# Autodesk Inventor assembly: Передача с помощью зубчатых ремней
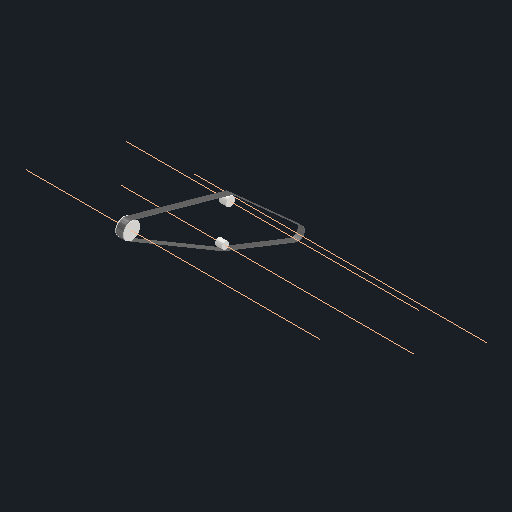
[picture p0: Inventor's stored thumbnail of the model, 512x512]
Saved by Autodesk Inventor 2024 (Build 280153000, 153)
## iProperties
ClientObjectVersion: 1
Created: 2023-09-26
Part Number: Передача с помощью зубчатых ремней
Document SubType Name: Assembly
Designer: user
Author: user
## Documents named in this file (5)
- D:\Docs\Robot\3d_v2\main_assembly\Мастер проектирования\Передача с помощью зубчатых ремней1.iam
- D:\Docs\Robot\3d_v2\main_assembly\Мастер проектирования\Зубчатый ремень1.ipt
- D:\Docs\Robot\3d_v2\main_assembly\Мастер проектирования\Шкив гладкий11.ipt
- D:\Docs\Robot\3d_v2\main_assembly\Мастер проектирования\Синхронный шкив21.ipt
- D:\Docs\Robot\3d_v2\main_assembly\Мастер проектирования\Шкив гладкий21.ipt
## Components (4 placed, 4 different names)
1. Зубчатый ремень:1 — Заподлицо:1, Совмещение:1, Заподлицо:2, Совмещение:2, Совмещение:3, Заподлицо:3, Совмещение:4
2. Шкив гладкий1:1 — Заподлицо:1, Совмещение:1
3. Синхронный шкив2:1 — Заподлицо:2, Совмещение:2, Совмещение:3
4. Шкив гладкий2:1 — Заподлицо:3, Совмещение:4
## Relationships (7: Mate 4, Flush 3)
- Заподлицо:1 [Flush]: Зубчатый ремень:1 ↔ Шкив гладкий1:1
- Совмещение:1 [Mate]: Зубчатый ремень:1 ↔ Шкив гладкий1:1
- Заподлицо:2 [Flush]: Зубчатый ремень:1 ↔ Синхронный шкив2:1
- Совмещение:2 [Mate]: Зубчатый ремень:1 ↔ Синхронный шкив2:1
- Совмещение:3 [Mate]: Зубчатый ремень:1 ↔ Синхронный шкив2:1
- Заподлицо:3 [Flush]: Зубчатый ремень:1 ↔ Шкив гладкий2:1
- Совмещение:4 [Mate]: Зубчатый ремень:1 ↔ Шкив гладкий2:1
